# Autodesk Inventor assembly: Conveyor
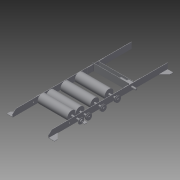
[picture p0: Inventor's stored thumbnail of the model, 180x180]
Saved by Autodesk Inventor 2015 (Build 190159000, 159)
## iProperties
Created: 2015-01-11
Part Number: Conveyor
Document SubType Name: Assembly
Designer: chapale16
Author: chapale16
## Documents named in this file (7)
- \\lhssvr02\Homedirs\Robotics Club\CAD Model 2015\CDR prep\Conveyor\Conveyor.iam
- \\lhssvr02\Homedirs\Robotics Club\CAD Model 2015\Box Beam Drive Base\Axle With single sprocket.iam
- \\lhssvr02\Homedirs\Robotics Club\CAD Model 2015\CDR prep\Conveyor\Double Sprocket Axle.iam
- \\lhssvr02\Homedirs\Robotics Club\CAD Model 2015\CDR prep\Conveyor\Conveyor Support_MIR2.ipt
- \\lhssvr02\Homedirs\Robotics Club\CAD Model 2015\CDR prep\Conveyor\Conveyor Support_MIR2_MIR.ipt
- \\lhssvr02\Homedirs\Robotics Club\CAD Model 2015\Game Components\The Tote Collector-Arms\P60 Gear Box.ipt
- \\lhssvr02\Homedirs\Robotics Club\CAD Model 2015\CDR prep\Conveyor\Conveyor Brace.ipt
## Components (9 placed, 6 different names)
1. Axle With single sprocket:1 [sub-assembly] — Mate:20
2. Double Sprocket Axle:1 [sub-assembly] — Mate:10
3. Double Sprocket Axle:2 [sub-assembly] — Mate:11
4. Conveyor Support_MIR2:1 — Flush:1, Flush:2, Mate:8, Mate:10, Mate:11, Mate:13, Mate:14, Mate:15, Angle:1, Flush:3, Flush:4, Mate:20
5. Conveyor Support_MIR2_MIR:1 — Flush:1, Flush:2, Mate:8, Mate:16, Mate:17
6. Double Sprocket Axle:3 [sub-assembly] — Mate:13
7. P60 Gear Box:2 — Mate:14, Mate:15, Angle:1, Mate:18, Mate:19
8. Conveyor Brace:1 — Flush:3, Mate:16, Mate:18
9. Conveyor Brace:2 — Flush:4, Mate:17, Mate:19
## Relationships (16: Mate 11, Flush 4, Angle 1)
- Flush:1: Conveyor Support_MIR2:1 ↔ Conveyor Support_MIR2_MIR:1
- Flush:2: Conveyor Support_MIR2:1 ↔ Conveyor Support_MIR2_MIR:1
- Mate:8 (304.8 mm): Conveyor Support_MIR2:1 ↔ Conveyor Support_MIR2_MIR:1
- Mate:10: Double Sprocket Axle:1 ↔ Conveyor Support_MIR2:1
- Mate:11: Double Sprocket Axle:2 ↔ Conveyor Support_MIR2:1
- Mate:13: Conveyor Support_MIR2:1 ↔ Double Sprocket Axle:3
- Mate:14: Conveyor Support_MIR2:1 ↔ P60 Gear Box:2
- Mate:15: Conveyor Support_MIR2:1 ↔ P60 Gear Box:2
- Angle:1 (0 deg): Conveyor Support_MIR2:1 ↔ P60 Gear Box:2
- Flush:3: Conveyor Support_MIR2:1 ↔ Conveyor Brace:1
- Flush:4: Conveyor Support_MIR2:1 ↔ Conveyor Brace:2
- Mate:16: Conveyor Support_MIR2_MIR:1 ↔ Conveyor Brace:1
- Mate:17: Conveyor Support_MIR2_MIR:1 ↔ Conveyor Brace:2
- Mate:18: P60 Gear Box:2 ↔ Conveyor Brace:1
- Mate:19: P60 Gear Box:2 ↔ Conveyor Brace:2
- Mate:20: Axle With single sprocket:1 ↔ Conveyor Support_MIR2:1
